# Autodesk Inventor assembly: 2924-1015-1000 assembly
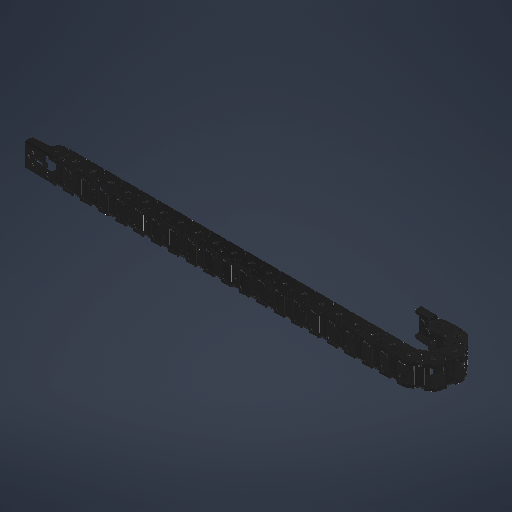
[picture p0: Inventor's stored thumbnail of the model, 512x512]
Saved by Autodesk Inventor 2026.2 (Build 302298000, 298)
## iProperties
Created: 2023-10-18
Part Number: 2924-1015-1000 assembly
Description: STEP AP203
Document SubType Name: Assembly
Designer: Kenji
Sending System: SolidWorks 2016
Preprocessor: SwSTEP 2.0
Title: 2924-1015-1000 assembly.STEP
Revision Number: ANY
## Documents named in this file (4)
- C:\Users\Kenji\Documents\GitHub\DiyCNC-\COTS-Parts\10x15-CarbleCarrierXAxis-2924-1015-1000.iam
- C:\Users\Kenji\Downloads\2924-1015-1000\2924-1015-1000 assembly\2924-1015-1000 assembly\2924-1015 End 1.ipt
- C:\Users\Kenji\Downloads\2924-1015-1000\2924-1015-1000 assembly\2924-1015-1000 assembly\2924-1015 link.ipt
- C:\Users\Kenji\Downloads\2924-1015-1000\2924-1015-1000 assembly\2924-1015-1000 assembly\2924-1015 End 2.ipt
## Components (26 placed, 10 different names)
1. 2924-1015 End 1_1 — Mate:1, Mate:2, Mate:3, Angle:1
2. 2924-1015 link_2 — Mate:1, Mate:2, Mate:3, Mate:4, Mate:5, Mate:6
3. 2924-1015 link_3 — Mate:10, Mate:11, Mate:12, Mate:13, Mate:14
4. 2924-1015 link_4 — Mate:4, Mate:5, Mate:6, Mate:7, Mate:8, Mate:9
5. 2924-1015 link_5 — Mate:7, Mate:8, Mate:9, Mate:10, Mate:11, Mate:12
6. 2924-1015 link_6 — Mate:13, Mate:14, Angle:1, Mate:15, Mate:16, Mate:17
7. 2924-1015 link_7 — Mate:15, Mate:16, Mate:17, Mate:18, Mate:19, Mate:20
8. 2924-1015 End 2:2 — Mate:21, Mate:22, Tangent:1
9. 2924-1015 link_8 — Mate:18, Mate:19, Mate:20
10. 2924-1015 link:58
11. 2924-1015 link:59
12. 2924-1015 link:60
13. 2924-1015 link:61
14. 2924-1015 link:62
15. 2924-1015 link:63
16. 2924-1015 link:64
17. 2924-1015 link:65
18. 2924-1015 link:66
19. 2924-1015 link:67
20. 2924-1015 link:68
21. 2924-1015 link:69
22. 2924-1015 link:70
23. 2924-1015 link:71
24. 2924-1015 link:72
25. 2924-1015 link:73
26. 2924-1015 link:74 — Mate:21, Mate:22, Tangent:1
## Component patterns: (18 elements, first: 2924-1015 link_8)
## Relationships (24: Mate 22, Angle 1, Tangent 1)
- Mate:1: 2924-1015 End 1_1 ↔ 2924-1015 link_2
- Mate:2: 2924-1015 End 1_1 ↔ 2924-1015 link_2
- Mate:3: 2924-1015 End 1_1 ↔ 2924-1015 link_2
- Mate:4: 2924-1015 link_2 ↔ 2924-1015 link_4
- Mate:5: 2924-1015 link_2 ↔ 2924-1015 link_4
- Mate:6: 2924-1015 link_2 ↔ 2924-1015 link_4
- Mate:7: 2924-1015 link_4 ↔ 2924-1015 link_5
- Mate:8: 2924-1015 link_4 ↔ 2924-1015 link_5
- Mate:9: 2924-1015 link_4 ↔ 2924-1015 link_5
- Mate:10: 2924-1015 link_3 ↔ 2924-1015 link_5
- Mate:11: 2924-1015 link_3 ↔ 2924-1015 link_5
- Mate:12: 2924-1015 link_3 ↔ 2924-1015 link_5
- Mate:13: 2924-1015 link_3 ↔ 2924-1015 link_6
- Mate:14: 2924-1015 link_3 ↔ 2924-1015 link_6
- Angle:1 (0 deg): 2924-1015 End 1_1 ↔ 2924-1015 link_6
- Mate:15: 2924-1015 link_6 ↔ 2924-1015 link_7
- Mate:16: 2924-1015 link_6 ↔ 2924-1015 link_7
- Mate:17: 2924-1015 link_6 ↔ 2924-1015 link_7
- Mate:18: 2924-1015 link_7 ↔ 2924-1015 link_8
- Mate:19: 2924-1015 link_7 ↔ 2924-1015 link_8
- Mate:20: 2924-1015 link_7 ↔ 2924-1015 link_8
- Mate:21: 2924-1015 End 2:2 ↔ 2924-1015 link:74
- Mate:22: 2924-1015 End 2:2 ↔ 2924-1015 link:74
- Tangent:1: 2924-1015 End 2:2 ↔ 2924-1015 link:74
